# Autodesk Inventor assembly: option 1 pit
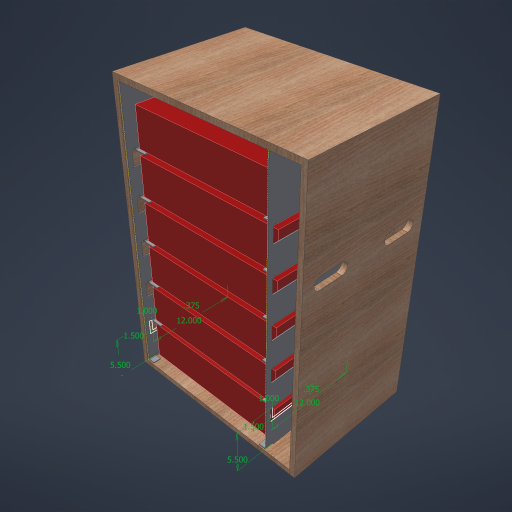
[picture p0: Inventor's stored thumbnail of the model, 512x512]
Saved by Autodesk Inventor 2023.4 (Build 274418000, 418)
## iProperties
Created: 2025-03-02
Part Number: option 1 pit
Document SubType Name: Assembly
Designer: brand
Author: brand
## Documents named in this file (5)
- C:\Users\brand\OneDrive\Documents\GitHub\robotics 23\2025-ReefScape---CAD\Pit\option 1 pit.iam
- C:\Users\brand\OneDrive\Documents\GitHub\robotics 23\2025-ReefScape---CAD\Pit\old battery cart.ipt
- C:\Users\brand\OneDrive\Documents\GitHub\robotics 23\2025-ReefScape---CAD\Pit\big craftsman.ipt
- C:\Users\brand\OneDrive\Documents\GitHub\robotics 23\2025-ReefScape---CAD\Pit\wall.ipt
- C:\Users\brand\OneDrive\Documents\GitHub\robotics 23\2025-ReefScape---CAD\Pit\wall2.ipt
## Components (9 placed, 4 different names)
1. old battery cart:1 — Mate:1, Mate:2, Mate:3, Mate:4, Mate:6, Mate:7, Mate:8
2. big craftsman:1 — Flush:1, Flush:6, Mate:1, Mate:2, Mate:5, Mate:9, Mate:11
3. big craftsman:2 — Flush:1, Flush:2, Flush:6, Flush:7, Mate:10
4. big craftsman:3 — Flush:2, Flush:3, Flush:7, Flush:8, Mate:12
5. big craftsman:4 — Flush:3, Flush:4, Flush:8, Flush:9, Mate:15
6. big craftsman:5 — Flush:4, Flush:5, Flush:9, Flush:10, Mate:14
7. big craftsman:6 — Flush:5, Flush:10, Mate:13
8. wall:1 — Mate:3, Mate:4, Mate:5
9. wall2:1 — Mate:6, Mate:7, Mate:8, Mate:9, Mate:10, Mate:11, Mate:12, Mate:13, Mate:14, Mate:15
## Relationships (25: Mate 15, Flush 10)
- Flush:1: big craftsman:1 ↔ big craftsman:2
- Flush:2: big craftsman:2 ↔ big craftsman:3
- Flush:3: big craftsman:3 ↔ big craftsman:4
- Flush:4: big craftsman:4 ↔ big craftsman:5
- Flush:5: big craftsman:5 ↔ big craftsman:6
- Flush:6: big craftsman:1 ↔ big craftsman:2
- Flush:7: big craftsman:2 ↔ big craftsman:3
- Flush:8: big craftsman:3 ↔ big craftsman:4
- Flush:9: big craftsman:4 ↔ big craftsman:5
- Flush:10: big craftsman:5 ↔ big craftsman:6
- Mate:1: old battery cart:1 ↔ big craftsman:1
- Mate:2: old battery cart:1 ↔ big craftsman:1
- Mate:3: old battery cart:1 ↔ wall:1
- Mate:4: old battery cart:1 ↔ wall:1
- Mate:5: big craftsman:1 ↔ wall:1
- Mate:6: old battery cart:1 ↔ wall2:1
- Mate:7: old battery cart:1 ↔ wall2:1
- Mate:8: old battery cart:1 ↔ wall2:1
- Mate:9 (6.35 mm): big craftsman:1 ↔ wall2:1
- Mate:10: big craftsman:2 ↔ wall2:1
- Mate:11: big craftsman:1 ↔ wall2:1
- Mate:12: big craftsman:3 ↔ wall2:1
- Mate:13: big craftsman:6 ↔ wall2:1
- Mate:14: big craftsman:5 ↔ wall2:1
- Mate:15: big craftsman:4 ↔ wall2:1
